# Autodesk Inventor assembly: box assembly
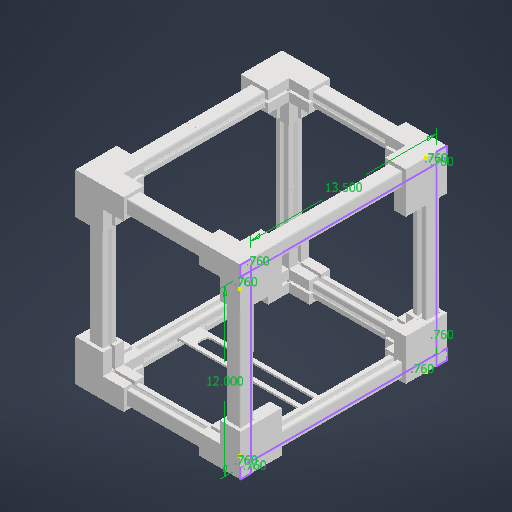
[picture p0: Inventor's stored thumbnail of the model, 512x512]
Saved by Autodesk Inventor 2026.2 (Build 302298000, 298)
## iProperties
Created: 2026-01-15
Part Number: box assembly
Document SubType Name: Assembly
Designer: dongr
Author: dongr
## Documents named in this file (10)
- C:\Users\dongr\OneDrive\Desktop\autodesk\box project\emitter case\box assembly.iam
- C:\Users\dongr\OneDrive\Desktop\autodesk\box project\emitter case\8020 skeleton\8020-1002-S X 6 male.ipt
- C:\Users\dongr\OneDrive\Desktop\autodesk\box project\emitter case\8020 skeleton\8020-1002-S X 6_5.ipt
- C:\Users\dongr\OneDrive\Desktop\autodesk\box project\emitter case\8020 skeleton\8020-1002-S X 5.ipt
- C:\Users\dongr\OneDrive\Desktop\autodesk\box project\emitter case\corner connector.ipt
- C:\Users\dongr\OneDrive\Desktop\autodesk\box project\emitter case\corner connector with rails (front right).ipt
- C:\Users\dongr\OneDrive\Desktop\autodesk\box project\emitter case\corner connector with rails (front left).ipt
- C:\Users\dongr\OneDrive\Desktop\autodesk\box project\emitter case\corner connector w rail (back).ipt
- C:\Users\dongr\OneDrive\Desktop\autodesk\box project\emitter case\corner support.ipt
- C:\Users\dongr\OneDrive\Desktop\autodesk\box project\emitter case\short slider.ipt
## Components (37 placed, 9 different names)
1. 8020-1002-S X 6 male:1 — Mate:4, Flush:7, Flush:8, Mate:7, Mate:9, Mate:10, Flush:11, Mate:75
2. 8020-1002-S X 6 male:2 — Flush:1, Flush:2, Mate:1, Mate:5, Flush:9
3. 8020-1002-S X 6 male:3 — Flush:5, Flush:6, Mate:3, Mate:15, Flush:14
4. 8020-1002-S X 6 male:4 — Flush:3, Flush:4, Mate:2, Mate:11, Mate:12, Flush:12
5. 8020-1002-S X 6_5:1 — Mate:4, Flush:7, Flush:8, Mate:8, Flush:10
6. 8020-1002-S X 6_5:2 — Flush:5, Flush:6, Mate:3, Mate:16, Mate:17
7. 8020-1002-S X 5:1 — Flush:3, Flush:4, Mate:2, Mate:18, Mate:19
8. 8020-1002-S X 5:2 — Flush:1, Flush:2, Mate:1, Mate:6, Mate:13, Mate:14, Flush:13
9. corner connector:1 — Mate:9, Mate:10, Flush:11, Mate:11, Mate:12, Flush:12, Mate:32, Mate:33, Mate:34, Mate:70, Mate:71
10. corner connector:2 — Mate:17, Mate:18, Mate:19, Mate:21, Mate:22, Mate:23, Mate:65, Mate:66, Mate:67
11. corner connector:3 — Mate:13, Mate:14, Flush:13, Mate:15, Mate:16, Flush:14, Mate:29, Mate:30, Mate:31, Mate:72, Mate:73
12. corner connector:4 — Mate:5, Mate:6, Flush:9, Mate:7, Mate:8, Flush:10, Mate:39, Mate:40, Mate:41, Mate:68, Mate:69
13. corner connector with rails (front right):1 — Mate:45, Mate:46, Mate:47, Mate:74
14. corner connector with rails (front left):1 — Mate:42, Mate:43, Mate:44, Mate:59, Mate:62, Mate:63
15. corner connector w rail (back):1 — Mate:24, Mate:25, Mate:26, Mate:55, Mate:57, Mate:58
16. corner connector w rail (back):2 — Mate:35, Mate:36, Mate:37, Mate:53, Mate:54
17. 8020-1002-S X 6 male:6 — Mate:28, Flush:19, Flush:20, Mate:42, Mate:43, Mate:44, Mate:60, Mate:64
18. 8020-1002-S X 6 male:7 — Mate:27, Flush:17, Flush:18, Mate:35, Mate:36, Mate:37, Mate:52
19. 8020-1002-S X 6 male:8 — Mate:20, Flush:15, Flush:16, Mate:22, Mate:23, Mate:24, Mate:25, Mate:26, Mate:56
20. 8020-1002-S X 5:3 — Mate:20, Flush:15, Flush:16, Mate:21
21. 8020-1002-S X 5:5 — Mate:27, Flush:17, Flush:18, Mate:32, Mate:33, Mate:34
22. 8020-1002-S X 5:6 — Mate:28, Flush:19, Flush:20, Mate:29, Mate:30, Mate:31
23. 8020-1002-S X 6 male:9 — Mate:38, Flush:21, Flush:22, Mate:39, Mate:40, Mate:41
24. 8020-1002-S X 6 male:10 — Mate:51, Flush:29, Flush:30
25. 8020-1002-S X 6 male:12 — Mate:48, Flush:23, Flush:24, Mate:58
26. 8020-1002-S X 6 male:13 — Mate:50, Flush:27, Flush:28, Flush:31
27. 8020-1002-S X 5:7 — Mate:38, Flush:21, Flush:22, Mate:45, Mate:46, Mate:47
28. 8020-1002-S X 5:8 — Mate:51, Flush:29, Flush:30, Mate:55, Mate:56, Mate:57
29. 8020-1002-S X 6_5:3 — Mate:48, Flush:23, Flush:24, Mate:59, Mate:60
30. 8020-1002-S X 6_5:4 — Mate:50, Flush:27, Flush:28, Mate:52, Flush:31, Mate:53, Mate:54
31. 8020-1002-S X 6 male:14 — Mate:61, Flush:32, Flush:33, Mate:63, Mate:64
32. 8020-1002-S X 5:9 — Mate:61, Flush:32, Flush:33, Mate:62
33. corner support:1 — Flush:34, Mate:70, Mate:71
34. corner support:2 — Flush:34, Flush:35, Mate:72, Mate:73
35. corner support:3 — Flush:35, Flush:36, Mate:68, Mate:69
36. corner support:4 — Flush:36, Mate:65, Mate:66, Mate:67
37. short slider:1 — Mate:74, Mate:75
## Relationships (108: Mate 74, Flush 34)
- Flush:1: 8020-1002-S X 6 male:2 ↔ 8020-1002-S X 5:2
- Flush:2: 8020-1002-S X 6 male:2 ↔ 8020-1002-S X 5:2
- Mate:1: 8020-1002-S X 6 male:2 ↔ 8020-1002-S X 5:2
- Flush:3: 8020-1002-S X 6 male:4 ↔ 8020-1002-S X 5:1
- Flush:4: 8020-1002-S X 6 male:4 ↔ 8020-1002-S X 5:1
- Mate:2: 8020-1002-S X 6 male:4 ↔ 8020-1002-S X 5:1
- Flush:5: 8020-1002-S X 6 male:3 ↔ 8020-1002-S X 6_5:2
- Flush:6: 8020-1002-S X 6 male:3 ↔ 8020-1002-S X 6_5:2
- Mate:3: 8020-1002-S X 6 male:3 ↔ 8020-1002-S X 6_5:2
- Mate:4: 8020-1002-S X 6 male:1 ↔ 8020-1002-S X 6_5:1
- Flush:7: 8020-1002-S X 6 male:1 ↔ 8020-1002-S X 6_5:1
- Flush:8: 8020-1002-S X 6 male:1 ↔ 8020-1002-S X 6_5:1
- Mate:5: 8020-1002-S X 6 male:2 ↔ corner connector:4
- Mate:6: 8020-1002-S X 5:2 ↔ corner connector:4
- Flush:9: 8020-1002-S X 6 male:2 ↔ corner connector:4
- Mate:7: 8020-1002-S X 6 male:1 ↔ corner connector:4
- Mate:8: 8020-1002-S X 6_5:1 ↔ corner connector:4
- Flush:10: 8020-1002-S X 6_5:1 ↔ corner connector:4
- Mate:9: 8020-1002-S X 6 male:1 ↔ corner connector:1
- Mate:10: 8020-1002-S X 6 male:1 ↔ corner connector:1
- Flush:11: 8020-1002-S X 6 male:1 ↔ corner connector:1
- Mate:11: 8020-1002-S X 6 male:4 ↔ corner connector:1
- Mate:12: 8020-1002-S X 6 male:4 ↔ corner connector:1
- Flush:12: 8020-1002-S X 6 male:4 ↔ corner connector:1
- Mate:13: 8020-1002-S X 5:2 ↔ corner connector:3
- Mate:14: 8020-1002-S X 5:2 ↔ corner connector:3
- Flush:13: 8020-1002-S X 5:2 ↔ corner connector:3
- Mate:15: 8020-1002-S X 6 male:3 ↔ corner connector:3
- Mate:16: 8020-1002-S X 6_5:2 ↔ corner connector:3
- Flush:14: 8020-1002-S X 6 male:3 ↔ corner connector:3
- Mate:17: 8020-1002-S X 6_5:2 ↔ corner connector:2
- Mate:18: 8020-1002-S X 5:1 ↔ corner connector:2
- Mate:19: 8020-1002-S X 5:1 ↔ corner connector:2
- Mate:20: 8020-1002-S X 6 male:8 ↔ 8020-1002-S X 5:3
- Flush:15: 8020-1002-S X 6 male:8 ↔ 8020-1002-S X 5:3
- Flush:16: 8020-1002-S X 6 male:8 ↔ 8020-1002-S X 5:3
- Mate:21: corner connector:2 ↔ 8020-1002-S X 5:3
- Mate:22: corner connector:2 ↔ 8020-1002-S X 6 male:8
- Mate:23: corner connector:2 ↔ 8020-1002-S X 6 male:8
- Mate:24: corner connector w rail (back):1 ↔ 8020-1002-S X 6 male:8
- Mate:25: corner connector w rail (back):1 ↔ 8020-1002-S X 6 male:8
- Mate:26: corner connector w rail (back):1 ↔ 8020-1002-S X 6 male:8
- Mate:27: 8020-1002-S X 6 male:7 ↔ 8020-1002-S X 5:5
- Flush:17: 8020-1002-S X 6 male:7 ↔ 8020-1002-S X 5:5
- Flush:18: 8020-1002-S X 6 male:7 ↔ 8020-1002-S X 5:5
- Mate:28: 8020-1002-S X 6 male:6 ↔ 8020-1002-S X 5:6
- Flush:19: 8020-1002-S X 6 male:6 ↔ 8020-1002-S X 5:6
- Flush:20: 8020-1002-S X 6 male:6 ↔ 8020-1002-S X 5:6
- Mate:29: corner connector:3 ↔ 8020-1002-S X 5:6
- Mate:30: corner connector:3 ↔ 8020-1002-S X 5:6
- Mate:31: corner connector:3 ↔ 8020-1002-S X 5:6
- Mate:32: corner connector:1 ↔ 8020-1002-S X 5:5
- Mate:33: corner connector:1 ↔ 8020-1002-S X 5:5
- Mate:34: corner connector:1 ↔ 8020-1002-S X 5:5
- Mate:35: corner connector w rail (back):2 ↔ 8020-1002-S X 6 male:7
- Mate:36: corner connector w rail (back):2 ↔ 8020-1002-S X 6 male:7
- Mate:37: corner connector w rail (back):2 ↔ 8020-1002-S X 6 male:7
- Mate:38: 8020-1002-S X 6 male:9 ↔ 8020-1002-S X 5:7
- Flush:21: 8020-1002-S X 6 male:9 ↔ 8020-1002-S X 5:7
- Flush:22: 8020-1002-S X 6 male:9 ↔ 8020-1002-S X 5:7
- Mate:39: corner connector:4 ↔ 8020-1002-S X 6 male:9
- Mate:40: corner connector:4 ↔ 8020-1002-S X 6 male:9
- Mate:41: corner connector:4 ↔ 8020-1002-S X 6 male:9
- Mate:42: corner connector with rails (front left):1 ↔ 8020-1002-S X 6 male:6
- Mate:43: corner connector with rails (front left):1 ↔ 8020-1002-S X 6 male:6
- Mate:44: corner connector with rails (front left):1 ↔ 8020-1002-S X 6 male:6
- Mate:45: corner connector with rails (front right):1 ↔ 8020-1002-S X 5:7
- Mate:46: corner connector with rails (front right):1 ↔ 8020-1002-S X 5:7
- Mate:47: corner connector with rails (front right):1 ↔ 8020-1002-S X 5:7
- Mate:48: 8020-1002-S X 6 male:12 ↔ 8020-1002-S X 6_5:3
- Flush:23: 8020-1002-S X 6 male:12 ↔ 8020-1002-S X 6_5:3
- Flush:24: 8020-1002-S X 6 male:12 ↔ 8020-1002-S X 6_5:3
- Mate:50: 8020-1002-S X 6 male:13 ↔ 8020-1002-S X 6_5:4
- Flush:27: 8020-1002-S X 6 male:13 ↔ 8020-1002-S X 6_5:4
- Flush:28: 8020-1002-S X 6 male:13 ↔ 8020-1002-S X 6_5:4
- Mate:51: 8020-1002-S X 6 male:10 ↔ 8020-1002-S X 5:8
- Flush:29: 8020-1002-S X 6 male:10 ↔ 8020-1002-S X 5:8
- Flush:30: 8020-1002-S X 6 male:10 ↔ 8020-1002-S X 5:8
- Mate:52: 8020-1002-S X 6 male:7 ↔ 8020-1002-S X 6_5:4
- Flush:31: 8020-1002-S X 6 male:13 ↔ 8020-1002-S X 6_5:4
- Mate:53: corner connector w rail (back):2 ↔ 8020-1002-S X 6_5:4
- Mate:54: corner connector w rail (back):2 ↔ 8020-1002-S X 6_5:4
- Mate:55: corner connector w rail (back):1 ↔ 8020-1002-S X 5:8
- Mate:56: 8020-1002-S X 6 male:8 ↔ 8020-1002-S X 5:8
- Mate:57: corner connector w rail (back):1 ↔ 8020-1002-S X 5:8
- Mate:58: corner connector w rail (back):1 ↔ 8020-1002-S X 6 male:12
- Mate:59: corner connector with rails (front left):1 ↔ 8020-1002-S X 6_5:3
- Mate:60: 8020-1002-S X 6 male:6 ↔ 8020-1002-S X 6_5:3
- Mate:61: 8020-1002-S X 6 male:14 ↔ 8020-1002-S X 5:9
- Flush:32: 8020-1002-S X 6 male:14 ↔ 8020-1002-S X 5:9
- Flush:33: 8020-1002-S X 6 male:14 ↔ 8020-1002-S X 5:9
- Mate:62: corner connector with rails (front left):1 ↔ 8020-1002-S X 5:9
- Mate:63: corner connector with rails (front left):1 ↔ 8020-1002-S X 6 male:14
- Mate:64: 8020-1002-S X 6 male:6 ↔ 8020-1002-S X 6 male:14
- Flush:34: corner support:1 ↔ corner support:2
- Flush:35: corner support:2 ↔ corner support:3
- Flush:36: corner support:3 ↔ corner support:4
- Mate:65: corner connector:2 ↔ corner support:4
- Mate:66: corner connector:2 ↔ corner support:4
- Mate:67: corner connector:2 ↔ corner support:4
- Mate:68: corner connector:4 ↔ corner support:3
- Mate:69: corner connector:4 ↔ corner support:3
- Mate:70: corner connector:1 ↔ corner support:1
- Mate:71: corner connector:1 ↔ corner support:1
- Mate:72: corner connector:3 ↔ corner support:2
- Mate:73: corner connector:3 ↔ corner support:2
- Mate:74: corner connector with rails (front right):1 ↔ short slider:1
- Mate:75: 8020-1002-S X 6 male:1 ↔ short slider:1
